# Autodesk Inventor assembly: Stadio2
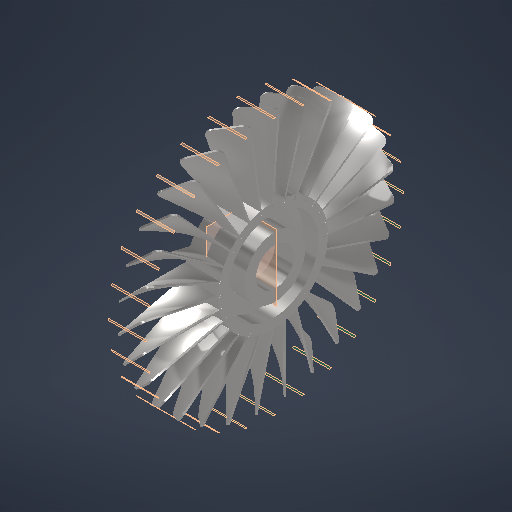
[picture p0: Inventor's stored thumbnail of the model, 512x512]
Saved by Autodesk Inventor 2026.2 (Build 302298010, 298A)
## iProperties
Created: 2026-04-23
Part Number: Stadio2
Document SubType Name: Assembly
Designer: Yan
Author: Yan
## Documents named in this file (3)
- C:\Users\Yan\Desktop\Turbina\Stadio2.iam
- C:\Users\Yan\Desktop\Turbina\DiscoPaleSatdio2-DimensioniAprossimate.ipt
- C:\Users\Yan\Desktop\Turbina\PalaStadio2.ipt
## Components (29 placed, 2 different names)
1. DiscoPaleSatdio2-DimensioniAprossimate:1 — Mate:1, Mate:2, Mate:3, Mate:4, Mate:5, Mate:6, Mate:7, Mate:8, Mate:9, Mate:10, Mate:11, Mate:12, Mate:13, Mate:14, Mate:15, Mate:16, Mate:17, Mate:18, Mate:19, Mate:20, Mate:21, Mate:22, Mate:23, Mate:24, Mate:25, Mate:26, Mate:27, Mate:28, Mate:29, Mate:30, Flush:1, Mate:31, Mate:32, Flush:2, Mate:33, Mate:34, Mate:35, Mate:36, Mate:37, Mate:38, Mate:39, Mate:40, Mate:41, Flush:3, Mate:42, Mate:43, Mate:44, Mate:45, Mate:46, Mate:47, Mate:48, Mate:49, Mate:50, Mate:51, Mate:52, Mate:53, Mate:54, Mate:55, Mate:56, Flush:4, Flush:5, Flush:6, Flush:7, Flush:8, Flush:13, Flush:14
2. PalaStadio2:1 — Mate:1, Mate:2, Flush:5, Flush:6, Flush:11, Flush:35
3. PalaStadio2:2 — Mate:3, Mate:4, Flush:4, Flush:7, Flush:10, Flush:34
4. PalaStadio2:3 — Mate:5, Mate:6, Flush:9, Flush:33
5. PalaStadio2:4 — Mate:7, Mate:8, Flush:8, Flush:9, Flush:10, Flush:11, Flush:12, Flush:32
6. PalaStadio2:5 — Mate:10, Mate:55, Flush:30
7. PalaStadio2:6 — Mate:9, Mate:56, Flush:31
8. PalaStadio2:7 — Mate:13, Mate:52, Flush:27
9. PalaStadio2:8 — Mate:14, Mate:51, Flush:26
10. PalaStadio2:9 — Mate:11, Mate:54, Flush:29
11. PalaStadio2:10 — Mate:12, Mate:53, Flush:28
12. PalaStadio2:11 — Mate:19, Mate:46, Flush:21
13. PalaStadio2:12 — Mate:18, Mate:47, Flush:22
14. PalaStadio2:13 — Mate:17, Mate:48, Flush:23
15. PalaStadio2:14 — Mate:16, Mate:49, Flush:24
16. PalaStadio2:15 — Mate:15, Mate:50, Flush:25
17. PalaStadio2:16 — Mate:26, Mate:27, Flush:15
18. PalaStadio2:17 — Mate:24, Mate:25, Flush:16
19. PalaStadio2:18 — Mate:23, Mate:42, Flush:17
20. PalaStadio2:19 — Mate:21, Mate:44, Flush:19
21. PalaStadio2:20 — Mate:20, Mate:45, Flush:20
22. PalaStadio2:21 — Mate:33, Mate:34, Flush:13, Flush:39
23. PalaStadio2:22 — Mate:36, Mate:41, Flush:3, Flush:38
24. PalaStadio2:23 — Mate:37, Mate:40, Flush:37
25. PalaStadio2:24 — Mate:38, Mate:39, Flush:12, Flush:36
26. PalaStadio2:25 — Mate:22, Mate:43, Flush:18
27. PalaStadio2:26 — Mate:32, Flush:2, Mate:35, Flush:40
28. PalaStadio2:27 — Mate:30, Flush:1, Mate:31, Flush:41
29. PalaStadio2:28 — Mate:28, Mate:29, Flush:14, Flush:15, Flush:16, Flush:17, Flush:18, Flush:19, Flush:20, Flush:21, Flush:22, Flush:23, Flush:24, Flush:25, Flush:26, Flush:27, Flush:28, Flush:29, Flush:30, Flush:31, Flush:32, Flush:33, Flush:34, Flush:35, Flush:36, Flush:37, Flush:38, Flush:39, Flush:40, Flush:41
## Relationships (97: Mate 56, Flush 41)
- Mate:1: DiscoPaleSatdio2-DimensioniAprossimate:1 ↔ PalaStadio2:1
- Mate:2: DiscoPaleSatdio2-DimensioniAprossimate:1 ↔ PalaStadio2:1
- Mate:3: DiscoPaleSatdio2-DimensioniAprossimate:1 ↔ PalaStadio2:2
- Mate:4: DiscoPaleSatdio2-DimensioniAprossimate:1 ↔ PalaStadio2:2
- Mate:5: DiscoPaleSatdio2-DimensioniAprossimate:1 ↔ PalaStadio2:3
- Mate:6: DiscoPaleSatdio2-DimensioniAprossimate:1 ↔ PalaStadio2:3
- Mate:7: DiscoPaleSatdio2-DimensioniAprossimate:1 ↔ PalaStadio2:4
- Mate:8: DiscoPaleSatdio2-DimensioniAprossimate:1 ↔ PalaStadio2:4
- Mate:9: DiscoPaleSatdio2-DimensioniAprossimate:1 ↔ PalaStadio2:6
- Mate:10: DiscoPaleSatdio2-DimensioniAprossimate:1 ↔ PalaStadio2:5
- Mate:11: DiscoPaleSatdio2-DimensioniAprossimate:1 ↔ PalaStadio2:9
- Mate:12: DiscoPaleSatdio2-DimensioniAprossimate:1 ↔ PalaStadio2:10
- Mate:13: DiscoPaleSatdio2-DimensioniAprossimate:1 ↔ PalaStadio2:7
- Mate:14: DiscoPaleSatdio2-DimensioniAprossimate:1 ↔ PalaStadio2:8
- Mate:15: DiscoPaleSatdio2-DimensioniAprossimate:1 ↔ PalaStadio2:15
- Mate:16: DiscoPaleSatdio2-DimensioniAprossimate:1 ↔ PalaStadio2:14
- Mate:17: DiscoPaleSatdio2-DimensioniAprossimate:1 ↔ PalaStadio2:13
- Mate:18: DiscoPaleSatdio2-DimensioniAprossimate:1 ↔ PalaStadio2:12
- Mate:19: DiscoPaleSatdio2-DimensioniAprossimate:1 ↔ PalaStadio2:11
- Mate:20: DiscoPaleSatdio2-DimensioniAprossimate:1 ↔ PalaStadio2:20
- Mate:21: DiscoPaleSatdio2-DimensioniAprossimate:1 ↔ PalaStadio2:19
- Mate:22: DiscoPaleSatdio2-DimensioniAprossimate:1 ↔ PalaStadio2:25
- Mate:23: DiscoPaleSatdio2-DimensioniAprossimate:1 ↔ PalaStadio2:18
- Mate:24: DiscoPaleSatdio2-DimensioniAprossimate:1 ↔ PalaStadio2:17
- Mate:25: DiscoPaleSatdio2-DimensioniAprossimate:1 ↔ PalaStadio2:17
- Mate:26: DiscoPaleSatdio2-DimensioniAprossimate:1 ↔ PalaStadio2:16
- Mate:27: DiscoPaleSatdio2-DimensioniAprossimate:1 ↔ PalaStadio2:16
- Mate:28: DiscoPaleSatdio2-DimensioniAprossimate:1 ↔ PalaStadio2:28
- Mate:29: DiscoPaleSatdio2-DimensioniAprossimate:1 ↔ PalaStadio2:28
- Mate:30: DiscoPaleSatdio2-DimensioniAprossimate:1 ↔ PalaStadio2:27
- Flush:1: DiscoPaleSatdio2-DimensioniAprossimate:1 ↔ PalaStadio2:27
- Mate:31: DiscoPaleSatdio2-DimensioniAprossimate:1 ↔ PalaStadio2:27
- Mate:32: DiscoPaleSatdio2-DimensioniAprossimate:1 ↔ PalaStadio2:26
- Flush:2: DiscoPaleSatdio2-DimensioniAprossimate:1 ↔ PalaStadio2:26
- Mate:33: DiscoPaleSatdio2-DimensioniAprossimate:1 ↔ PalaStadio2:21
- Mate:34: DiscoPaleSatdio2-DimensioniAprossimate:1 ↔ PalaStadio2:21
- Mate:35: DiscoPaleSatdio2-DimensioniAprossimate:1 ↔ PalaStadio2:26
- Mate:36: DiscoPaleSatdio2-DimensioniAprossimate:1 ↔ PalaStadio2:22
- Mate:37: DiscoPaleSatdio2-DimensioniAprossimate:1 ↔ PalaStadio2:23
- Mate:38: DiscoPaleSatdio2-DimensioniAprossimate:1 ↔ PalaStadio2:24
- Mate:39: DiscoPaleSatdio2-DimensioniAprossimate:1 ↔ PalaStadio2:24
- Mate:40: DiscoPaleSatdio2-DimensioniAprossimate:1 ↔ PalaStadio2:23
- Mate:41: DiscoPaleSatdio2-DimensioniAprossimate:1 ↔ PalaStadio2:22
- Flush:3: DiscoPaleSatdio2-DimensioniAprossimate:1 ↔ PalaStadio2:22
- Mate:42: DiscoPaleSatdio2-DimensioniAprossimate:1 ↔ PalaStadio2:18
- Mate:43: DiscoPaleSatdio2-DimensioniAprossimate:1 ↔ PalaStadio2:25
- Mate:44: DiscoPaleSatdio2-DimensioniAprossimate:1 ↔ PalaStadio2:19
- Mate:45: DiscoPaleSatdio2-DimensioniAprossimate:1 ↔ PalaStadio2:20
- Mate:46: DiscoPaleSatdio2-DimensioniAprossimate:1 ↔ PalaStadio2:11
- Mate:47: DiscoPaleSatdio2-DimensioniAprossimate:1 ↔ PalaStadio2:12
- Mate:48: DiscoPaleSatdio2-DimensioniAprossimate:1 ↔ PalaStadio2:13
- Mate:49: DiscoPaleSatdio2-DimensioniAprossimate:1 ↔ PalaStadio2:14
- Mate:50: DiscoPaleSatdio2-DimensioniAprossimate:1 ↔ PalaStadio2:15
- Mate:51: DiscoPaleSatdio2-DimensioniAprossimate:1 ↔ PalaStadio2:8
- Mate:52: DiscoPaleSatdio2-DimensioniAprossimate:1 ↔ PalaStadio2:7
- Mate:53: DiscoPaleSatdio2-DimensioniAprossimate:1 ↔ PalaStadio2:10
- Mate:54: DiscoPaleSatdio2-DimensioniAprossimate:1 ↔ PalaStadio2:9
- Mate:55: DiscoPaleSatdio2-DimensioniAprossimate:1 ↔ PalaStadio2:5
- Mate:56: DiscoPaleSatdio2-DimensioniAprossimate:1 ↔ PalaStadio2:6
- Flush:4: DiscoPaleSatdio2-DimensioniAprossimate:1 ↔ PalaStadio2:2
- Flush:5: DiscoPaleSatdio2-DimensioniAprossimate:1 ↔ PalaStadio2:1
- Flush:6: DiscoPaleSatdio2-DimensioniAprossimate:1 ↔ PalaStadio2:1
- Flush:7: DiscoPaleSatdio2-DimensioniAprossimate:1 ↔ PalaStadio2:2
- Flush:8: DiscoPaleSatdio2-DimensioniAprossimate:1 ↔ PalaStadio2:4
- Flush:9: PalaStadio2:3 ↔ PalaStadio2:4
- Flush:10: PalaStadio2:2 ↔ PalaStadio2:4
- Flush:11: PalaStadio2:1 ↔ PalaStadio2:4
- Flush:12: PalaStadio2:4 ↔ PalaStadio2:24
- Flush:13: DiscoPaleSatdio2-DimensioniAprossimate:1 ↔ PalaStadio2:21
- Flush:14: DiscoPaleSatdio2-DimensioniAprossimate:1 ↔ PalaStadio2:28
- Flush:15: PalaStadio2:16 ↔ PalaStadio2:28
- Flush:16: PalaStadio2:17 ↔ PalaStadio2:28
- Flush:17: PalaStadio2:18 ↔ PalaStadio2:28
- Flush:18: PalaStadio2:25 ↔ PalaStadio2:28
- Flush:19: PalaStadio2:19 ↔ PalaStadio2:28
- Flush:20: PalaStadio2:20 ↔ PalaStadio2:28
- Flush:21: PalaStadio2:11 ↔ PalaStadio2:28
- Flush:22: PalaStadio2:12 ↔ PalaStadio2:28
- Flush:23: PalaStadio2:13 ↔ PalaStadio2:28
- Flush:24: PalaStadio2:14 ↔ PalaStadio2:28
- Flush:25: PalaStadio2:15 ↔ PalaStadio2:28
- Flush:26: PalaStadio2:8 ↔ PalaStadio2:28
- Flush:27: PalaStadio2:7 ↔ PalaStadio2:28
- Flush:28: PalaStadio2:10 ↔ PalaStadio2:28
- Flush:29: PalaStadio2:9 ↔ PalaStadio2:28
- Flush:30: PalaStadio2:5 ↔ PalaStadio2:28
- Flush:31: PalaStadio2:6 ↔ PalaStadio2:28
- Flush:32: PalaStadio2:4 ↔ PalaStadio2:28
- Flush:33: PalaStadio2:3 ↔ PalaStadio2:28
- Flush:34: PalaStadio2:2 ↔ PalaStadio2:28
- Flush:35: PalaStadio2:1 ↔ PalaStadio2:28
- Flush:36: PalaStadio2:24 ↔ PalaStadio2:28
- Flush:37: PalaStadio2:23 ↔ PalaStadio2:28
- Flush:38: PalaStadio2:22 ↔ PalaStadio2:28
- Flush:39: PalaStadio2:21 ↔ PalaStadio2:28
- Flush:40: PalaStadio2:26 ↔ PalaStadio2:28
- Flush:41: PalaStadio2:27 ↔ PalaStadio2:28
